# Autodesk Inventor assembly: BBP
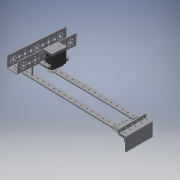
[picture p0: Inventor's stored thumbnail of the model, 180x180]
Saved by Autodesk Inventor 2016 (Build 200138000, 138)
## iProperties
Created: 2016-09-30
Part Number: BBP
Document SubType Name: Assembly
Designer: Delta
Author: Delta
## Documents named in this file (9)
- C:\Robotics\2016-17_CAD\BBP.iam
- C:\Robotics\COTSParts\Tetrix\Tetrix channel 160mm.ipt
- C:\Robotics\COTSParts\Tetrix\Tetrix flat bar 288mm.ipt
- C:\Robotics\COTSParts\Tetrix\Tetrix bracket - single servo.ipt
- C:\Robotics\COTSParts\Actobotics\585 parts\585382.ipt
- C:\Robotics\COTSParts\Tetrix\Tetrix servo 180.ipt
- C:\Robotics\2015-16_CAD\Part5.ipt
- C:\Robotics\2015-16_CAD\Part6.ipt
- C:\Robotics\2015-16_CAD\Tetrix angle 144mm_3in.ipt
## Components (10 placed, 8 different names)
1. Tetrix channel 160mm:2 — Insert:1, Insert:2, Insert:3, Insert:8
2. Tetrix flat bar 288mm:1 — Insert:1, Insert:6
3. Tetrix flat bar 288mm:2 — Insert:7
4. Tetrix bracket - single servo:1 — Insert:2, Insert:3, Mate:1, Flush:1, Flush:2
5. Tetrix servo 180:1 — Mate:1, Flush:1, Flush:2
6. 585382:5 — Insert:6, Insert:7, Insert:9
7. Part5:1 — Insert:8
8. Part6:1 — Mate:2, Flush:5, Flush:6
9. Tetrix angle 144mm_3in:1 — Flush:3, Flush:4, Insert:9
10. Tetrix angle 144mm_3in:2 — Flush:3, Flush:4, Mate:2, Flush:5, Flush:6
## Relationships (15: Insert 7, Flush 6, Mate 2)
- Insert:1 (25.4 mm): Tetrix channel 160mm:2 ↔ Tetrix flat bar 288mm:1
- Insert:2: Tetrix channel 160mm:2 ↔ Tetrix bracket - single servo:1
- Insert:3: Tetrix channel 160mm:2 ↔ Tetrix bracket - single servo:1
- Mate:1 (5.3594 mm): Tetrix bracket - single servo:1 ↔ Tetrix servo 180:1
- Flush:1: Tetrix bracket - single servo:1 ↔ Tetrix servo 180:1
- Flush:2: Tetrix bracket - single servo:1 ↔ Tetrix servo 180:1
- Insert:6: Tetrix flat bar 288mm:1 ↔ 585382:5
- Insert:7: Tetrix flat bar 288mm:2 ↔ 585382:5
- Insert:8: Tetrix channel 160mm:2 ↔ Part5:1
- Flush:3: Tetrix angle 144mm_3in:1 ↔ Tetrix angle 144mm_3in:2
- Flush:4: Tetrix angle 144mm_3in:1 ↔ Tetrix angle 144mm_3in:2
- Mate:2: Part6:1 ↔ Tetrix angle 144mm_3in:2
- Flush:5: Part6:1 ↔ Tetrix angle 144mm_3in:2
- Flush:6: Part6:1 ↔ Tetrix angle 144mm_3in:2
- Insert:9: 585382:5 ↔ Tetrix angle 144mm_3in:1
